# Autodesk Inventor assembly: Eva_Voyager21
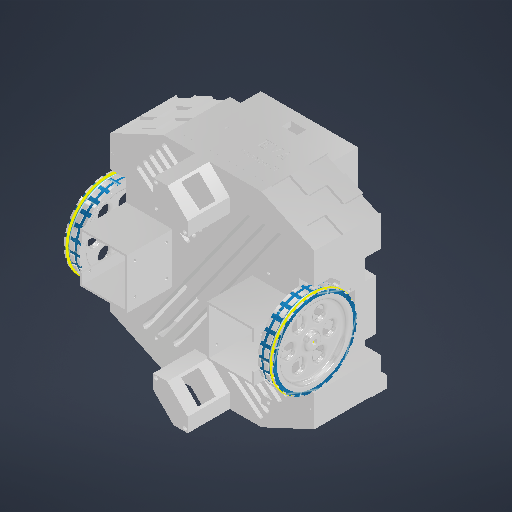
[picture p0: Inventor's stored thumbnail of the model, 512x512]
Saved by Autodesk Inventor 2026 (Build 300175000, 175)
## iProperties
Created: 2025-11-05
Part Number: Eva_Voyager21
Document SubType Name: Assembly
Designer: Nicolás De Bruijn
Author: Nicolás De Bruijn
## Documents named in this file (8)
- C:\Users\Nicolás De Bruijn\Desktop\Tecnologias Espaciales\Partes diseño 3D\Eva_Voyager21.iam
- C:\Users\Nicolás De Bruijn\Desktop\Tecnologias Espaciales\Partes diseño 3D\Aro_Rover.ipt
- C:\Users\Nicolás De Bruijn\Desktop\Tecnologias Espaciales\Partes diseño 3D\Caja_Antena.ipt
- C:\Users\Nicolás De Bruijn\Desktop\Tecnologias Espaciales\Partes diseño 3D\Caja_Bateria.ipt
- C:\Users\Nicolás De Bruijn\Desktop\Tecnologias Espaciales\Partes diseño 3D\Caja_Camara.ipt
- C:\Users\Nicolás De Bruijn\Desktop\Tecnologias Espaciales\Partes diseño 3D\Caja_Chasis.ipt
- C:\Users\Nicolás De Bruijn\Desktop\Tecnologias Espaciales\Partes diseño 3D\Chasis.ipt
- C:\Users\Nicolás De Bruijn\Desktop\Tecnologias Espaciales\Partes diseño 3D\Ruedas_Rover.ipt
## Components (9 placed, 7 different names)
1. Aro_Rover:1 — Rigid:2, Rigid:5
2. Caja_Antena:1 — Rotational:2
3. Caja_Bateria:1 — Rotational:1, Rotational:4
4. Caja_Chasis:1 — Rigid:1, Rotational:1, Rotational:2, Rotational:3, Rotational:4
5. Chasis:1 — Rigid:1, Rigid:4, Rigid:5
6. Ruedas_Rover:1 — Rigid:2
7. Aro_Rover:2 — Rigid:4
8. Ruedas_Rover:2
9. Caja_Camara:1 — Rotational:3
## Relationships (9: WeldJoint 5, RevoluteJoint 4)
- Rigid:1 [WeldJoint]: Caja_Chasis:1 ↔ Chasis:1
- Rigid:2 [WeldJoint]: Aro_Rover:1 ↔ Ruedas_Rover:1
- [WeldJoint]: Aro_Rover:2 ↔ Ruedas_Rover:2
- Rotational:1 [RevoluteJoint]: Caja_Bateria:1 ↔ Caja_Chasis:1
- Rotational:2 [RevoluteJoint]: Caja_Antena:1 ↔ Caja_Chasis:1
- Rigid:4 [WeldJoint] (2.54 mm): Chasis:1 ↔ Aro_Rover:2
- Rigid:5 [WeldJoint] (2.54 mm): Aro_Rover:1 ↔ Chasis:1
- Rotational:3 [RevoluteJoint]: Caja_Chasis:1 ↔ Caja_Camara:1
- Rotational:4 [RevoluteJoint]: Caja_Bateria:1 ↔ Caja_Chasis:1
## Named parameters: d2_d1 = 0 mm, Finish1_Area = 4361.55, Finish2_Area = 37.9173, Finish3_Area = 54.9301
note: some values were not read from the file. Shown as the stored number, unit unknown: "Finish1_Area", "Finish2_Area", "Finish3_Area".
